# Autodesk Inventor assembly: mascon-new
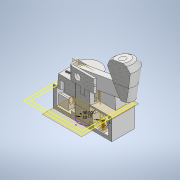
[picture p0: Inventor's stored thumbnail of the model, 180x180]
Saved by Autodesk Inventor 2021 (Build 250183000, 183)
## iProperties
Created: 2021-04-28
Part Number: mascon-new
Document SubType Name: Assembly
Designer: ben
Author: ben
## Documents named in this file (12)
- C:\Users\teh18\OneDrive\BVE Controller\r68-bve-mascon\mascon-new.iam
- C:\Users\teh18\OneDrive\BVE Controller\r68-bve-mascon\mascon.ipt
- C:\Users\teh18\OneDrive\BVE Controller\r68-bve-mascon\handle_base2.ipt
- C:\Users\teh18\OneDrive\BVE Controller\r68-bve-mascon\stl2\NotchPiston1.ipt
- C:\Users\teh18\OneDrive\BVE Controller\r68-bve-mascon\stl2\HandleBaseFiller.ipt
- C:\Users\teh18\OneDrive\BVE Controller\r68-bve-mascon\handle-stick.ipt
- C:\Users\teh18\OneDrive\BVE Controller\r68-bve-mascon\handle-sheath.ipt
- C:\Users\teh18\OneDrive\BVE Controller\r68-bve-mascon\stl2\Handle.iam
- C:\Users\teh18\OneDrive\BVE Controller\potentiometer-b10k-1.snapshot.2\PotentiometerB10K.ipt
- C:\Users\teh18\OneDrive\BVE Controller\r68-bve-mascon\PotHolder.ipt
- C:\Users\teh18\OneDrive\BVE Controller\r68-bve-mascon\stl2\HandleBaseFiller_MIR.ipt
- C:\Users\teh18\OneDrive\BVE Controller\r68-bve-mascon\handle-base\handle-base.iam
## Components (11 placed, 11 different names)
1. mascon:1 — Flush:3, Mate:3, Mate:4, Tangent:1, Mate:8, Mate:9
2. handle_base2:1 — Mate:7
3. NotchPiston1:1 — Flush:3
4. handle-sheath:1 — Mate:1, Mate:6
5. handle-stick:1 — Mate:1, Mate:6, Rotational:1
6. HandleBaseFiller:1
7. Handle:1 [sub-assembly]
8. PotentiometerB10K:1 — Mate:4, Tangent:1
9. PotHolder:1 — Mate:3
10. HandleBaseFiller_MIR:1
11. handle-base:1 [sub-assembly] — Mate:7, Mate:8, Mate:9, Rotational:1
## Relationships (10: Mate 7, Flush 1, Tangent 1, RevoluteJoint 1)
- Flush:3: mascon:1 ↔ NotchPiston1:1
- Mate:1: handle-sheath:1 ↔ handle-stick:1
- Mate:3: mascon:1 ↔ PotHolder:1
- Mate:4: mascon:1 ↔ PotentiometerB10K:1
- Tangent:1: mascon:1 ↔ PotentiometerB10K:1
- Mate:6: handle-sheath:1 ↔ handle-stick:1
- Mate:7: handle_base2:1 ↔ handle-base:1
- Mate:8: mascon:1 ↔ handle-base:1
- Mate:9: mascon:1 ↔ handle-base:1
- Rotational:1 [RevoluteJoint]: handle-stick:1 ↔ handle-base:1
